# Autodesk Inventor assembly: PnumaticActiveClimb-ver3-1111-2021
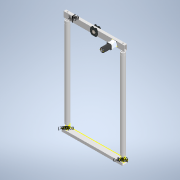
[picture p0: Inventor's stored thumbnail of the model, 180x180]
Saved by Autodesk Inventor 2021 (Build 250183000, 183)
## iProperties
Created: 2021-01-28
Part Number: PnumaticActiveClimb-ver3-1111-2021
Document SubType Name: Assembly
Designer: CMurray
Author: CMurray
## Documents named in this file (7)
- C:\Users\con_c_000\Documents\GitHub\RoboticsCad1111\PHRC CADD\2020 Infinite Recharge\2021 Infinite Recharge\Chassis\PnumaticActiveClimb-ver3-1111-2021.iam
- C:\Users\con_c_000\Documents\GitHub\RoboticsCad1111\PHRC CADD\2020 Infinite Recharge\Active Climb\Parts\2x1 16in Aluminum-ver1-1111-2020.ipt
- C:\Users\con_c_000\Documents\GitHub\RoboticsCad1111\PHRC CADD\Resources\VEXpro Resources\Versa Motion\VersaBlockKit-1111-2016.ipt
- C:\Users\con_c_000\Documents\GitHub\RoboticsCad1111\PHRC CADD\Resources\VEXpro Resources\Bearings\0.5inHexFlangedBearing(1.125inx0.313in)-1111-2016.ipt
- C:\Users\con_c_000\Documents\GitHub\RoboticsCad1111\PHRC CADD\Resources\VEXpro Resources\Motors\v2-VersaPlanetary-3in-1stage-with-775pro-20161031.iam
- C:\Users\con_c_000\Documents\GitHub\RoboticsCad1111\PHRC CADD\2020 Infinite Recharge\Lift\Parts\1.5_Bore_30in_Stroke_ROUND BODY AIR CYLINDER.iam
- C:\Users\con_c_000\Documents\GitHub\RoboticsCad1111\PHRC CADD\2020 Infinite Recharge\Lift\Assemblies\ClimbBase-1111-2020.iam
## Components (8 placed, 6 different names)
1. 2x1 16in Aluminum-ver1-1111-2020:1 — Rotational:1, Angle:1, Rotational:2, Angle:2, Cylindrical:21, Mate:24, Angle:26, Flush:7, Flush:8, Mate:25, Rotational:13
2. VersaBlockKit-1111-2016:1 — Rotational:1, Angle:1
3. VersaBlockKit-1111-2016:2 — Rotational:2, Angle:2
4. v2-VersaPlanetary-3in-1stage-with-775pro-20161031:1 [sub-assembly] — Cylindrical:21, Mate:24, Angle:26, Angle:27
5. 1.5_Bore_30in_Stroke_ROUND BODY AIR CYLINDER:3 [sub-assembly] — Flush:6
6. 1.5_Bore_30in_Stroke_ROUND BODY AIR CYLINDER:4 [sub-assembly] — Rotational:12, Flush:6
7. ClimbBase-1111-2020:2 [sub-assembly] — Rotational:12, Flush:7, Flush:8, Mate:25
8. 0.5inHexFlangedBearing(1.125inx0.313in)-1111-2016:9 — Rotational:13, Angle:27
## Relationships (15: RevoluteJoint 4, Angle 4, Flush 3, Mate 2, CylindricalJoint 1, Insert 1)
- Rotational:1 [RevoluteJoint]: 2x1 16in Aluminum-ver1-1111-2020:1 ↔ VersaBlockKit-1111-2016:1
- Angle:1 (0 deg): 2x1 16in Aluminum-ver1-1111-2020:1 ↔ VersaBlockKit-1111-2016:1
- Rotational:2 [RevoluteJoint]: 2x1 16in Aluminum-ver1-1111-2020:1 ↔ VersaBlockKit-1111-2016:2
- Angle:2 (0 deg): 2x1 16in Aluminum-ver1-1111-2020:1 ↔ VersaBlockKit-1111-2016:2
- Cylindrical:21: 2x1 16in Aluminum-ver1-1111-2020:1 ↔ v2-VersaPlanetary-3in-1stage-with-775pro-20161031:1
- Mate:24: 2x1 16in Aluminum-ver1-1111-2020:1 ↔ v2-VersaPlanetary-3in-1stage-with-775pro-20161031:1
- Angle:26 (0 deg): 2x1 16in Aluminum-ver1-1111-2020:1 ↔ v2-VersaPlanetary-3in-1stage-with-775pro-20161031:1
- [Insert]: 1.5_Bore_30in_Stroke_ROUND BODY AIR CYLINDER:3 ↔ ClimbBase-1111-2020:2
- Rotational:12 [RevoluteJoint]: 1.5_Bore_30in_Stroke_ROUND BODY AIR CYLINDER:4 ↔ ClimbBase-1111-2020:2
- Flush:6: 1.5_Bore_30in_Stroke_ROUND BODY AIR CYLINDER:3 ↔ 1.5_Bore_30in_Stroke_ROUND BODY AIR CYLINDER:4
- Flush:7: 2x1 16in Aluminum-ver1-1111-2020:1 ↔ ClimbBase-1111-2020:2
- Flush:8: 2x1 16in Aluminum-ver1-1111-2020:1 ↔ ClimbBase-1111-2020:2
- Mate:25 (889.635 mm): 2x1 16in Aluminum-ver1-1111-2020:1 ↔ ClimbBase-1111-2020:2
- Rotational:13 [RevoluteJoint]: 2x1 16in Aluminum-ver1-1111-2020:1 ↔ 0.5inHexFlangedBearing(1.125inx0.313in)-1111-2016:9
- Angle:27 (90 deg): v2-VersaPlanetary-3in-1stage-with-775pro-20161031:1 ↔ 0.5inHexFlangedBearing(1.125inx0.313in)-1111-2016:9
